# Autodesk Inventor assembly: PDM35E247-BS0802-1.5-4-40-001
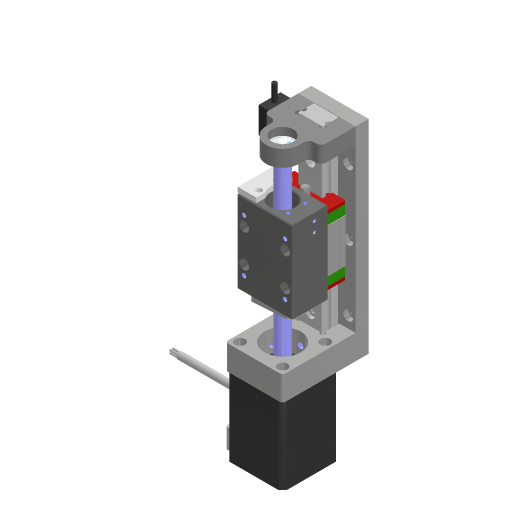
[picture p0: Inventor's stored thumbnail of the model, 512x512]
Saved by Autodesk Inventor 2023 (Build 270158000, 158)
## iProperties
Company: ZWCAD Software Co.
Created: 2026-04-09
Part Number: PDM35E247-BS0802-1.5-4-40-001
Description: This file contains a STEP AP42 implementation
Document SubType Name: Assembly
Designer: ferrerx
Sending System: ZW3D to STEP translator
Preprocessor: Version 1.0
Title: PDM35E247-BS0802-1.5-4-40-001.stp
Revision Number: ANYUNSPECIFIED
## Documents named in this file (16)
- C:\Users\ferrerx\The Francis Crick Dropbox\MakingLab\Projects\MSTP00412 - Linear cell stretcher\LMD14S18BAB15-040.iam
- C:\Users\ferrerx\The Francis Crick Dropbox\MakingLab\Projects\MSTP00412 - Linear cell stretcher\16-35-901.ipt
- C:\Users\ferrerx\The Francis Crick Dropbox\MakingLab\Projects\MSTP00412 - Linear cell stretcher\28-35-001.iam
- C:\Users\ferrerx\The Francis Crick Dropbox\MakingLab\Projects\MSTP00412 - Linear cell stretcher\16-35-902.ipt
- C:\Users\ferrerx\The Francis Crick Dropbox\MakingLab\Projects\MSTP00412 - Linear cell stretcher\16-42-914.ipt
- C:\Users\ferrerx\The Francis Crick Dropbox\MakingLab\Projects\MSTP00412 - Linear cell stretcher\12-015.ipt
- C:\Users\ferrerx\The Francis Crick Dropbox\MakingLab\Projects\MSTP00412 - Linear cell stretcher\03-42-914.ipt
- C:\Users\ferrerx\The Francis Crick Dropbox\MakingLab\Projects\MSTP00412 - Linear cell stretcher\03-42-916.ipt
- C:\Users\ferrerx\The Francis Crick Dropbox\MakingLab\Projects\MSTP00412 - Linear cell stretcher\09-28-002.ipt
- C:\Users\ferrerx\The Francis Crick Dropbox\MakingLab\Projects\MSTP00412 - Linear cell stretcher\11-003.ipt
- C:\Users\ferrerx\The Francis Crick Dropbox\MakingLab\Projects\MSTP00412 - Linear cell stretcher\16-35-903.ipt
- C:\Users\ferrerx\The Francis Crick Dropbox\MakingLab\Projects\MSTP00412 - Linear cell stretcher\B35E247-0-1.5-4-STD.ipt
- C:\Users\ferrerx\The Francis Crick Dropbox\MakingLab\Projects\MSTP00412 - Linear cell stretcher\16-35-904.ipt
- C:\Users\ferrerx\The Francis Crick Dropbox\MakingLab\Projects\MSTP00412 - Linear cell stretcher\12-004.ipt
- C:\Users\ferrerx\The Francis Crick Dropbox\MakingLab\Projects\MSTP00412 - Linear cell stretcher\21-42-903.ipt
- C:\Users\ferrerx\The Francis Crick Dropbox\MakingLab\Projects\MSTP00412 - Linear cell stretcher\Beam breaker.ipt
## Components (16 placed, 15 different names)
1. 16-35-901 — Mate:13, Mate:14, Mate:19, Mate:26
2. 28-35-001 [sub-assembly] — Mate:15, Mate:16, Mate:17, Mate:18
3. 16-35-902 — Mate:1, Mate:2, Mate:3, Mate:4, Flush:1, Mate:20, Mate:21, Mate:22
4. 16-42-914 — Mate:9, Mate:10, Mate:11, Mate:15, Mate:16, Mate:17, Mate:23, Mate:24, Mate:27, Mate:28, Mate:29
5. 03-42-914 — Mate:5, Mate:6, Mate:7, Mate:9, Mate:12
6. 03-42-916 — Mate:10, Mate:11
7. 09-28-002 — Mate:2, Mate:6, Flush:1, Mate:8
8. 11-003 — Mate:5, Mate:7, Mate:8
9. 16-35-903 — Mate:1, Mate:3, Mate:4, Mate:18, Mate:19
10. B35E247-0-1 — Mate:12, Mate:13, Mate:14, Mate:26
11. 16-35-904 — Mate:25
12. 12-004 — Mate:24, Mate:25
13. 12-004:1 — Mate:23
14. 21-42-903 — Mate:20, Mate:21, Mate:22
15. 12-015:4
16. Beam breaker:1 — Mate:27, Mate:28, Mate:29
## Relationships (30: Mate 29, Flush 1)
- Mate:1: 16-35-902 ↔ 16-35-903
- Mate:2: 16-35-902 ↔ 09-28-002
- Mate:3: 16-35-902 ↔ 16-35-903
- Mate:4: 16-35-902 ↔ 16-35-903
- Mate:5: 03-42-914 ↔ 11-003
- Mate:6: 03-42-914 ↔ 09-28-002
- Mate:7: 03-42-914 ↔ 11-003
- Flush:1: 16-35-902 ↔ 09-28-002
- Mate:8: 09-28-002 ↔ 11-003
- Mate:9: 16-42-914 ↔ 03-42-914
- Mate:10: 16-42-914 ↔ 03-42-916
- Mate:11: 16-42-914 ↔ 03-42-916
- Mate:12: 03-42-914 ↔ B35E247-0-1
- Mate:13: 16-35-901 ↔ B35E247-0-1
- Mate:14: 16-35-901 ↔ B35E247-0-1
- Mate:15: 28-35-001 ↔ 16-42-914
- Mate:16: 28-35-001 ↔ 16-42-914
- Mate:17: 28-35-001 ↔ 16-42-914
- Mate:18: 28-35-001 ↔ 16-35-903
- Mate:19: 16-35-901 ↔ 16-35-903
- Mate:20: 16-35-902 ↔ 21-42-903
- Mate:21: 16-35-902 ↔ 21-42-903
- Mate:22: 16-35-902 ↔ 21-42-903
- Mate:23: 16-42-914 ↔ 12-004:1
- Mate:24: 16-42-914 ↔ 12-004
- Mate:25: 16-35-904 ↔ 12-004
- Mate:26: 16-35-901 ↔ B35E247-0-1
- Mate:27: 16-42-914 ↔ Beam breaker:1
- Mate:28: 16-42-914 ↔ Beam breaker:1
- Mate:29: 16-42-914 ↔ Beam breaker:1
